# Autodesk Inventor assembly: 2024-000
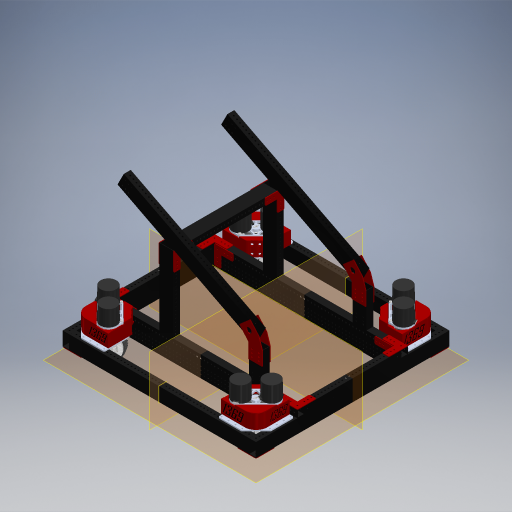
[picture p0: Inventor's stored thumbnail of the model, 512x512]
Saved by Autodesk Inventor 2024.2 (Build 282272000, 272)
## iProperties
Created: 2024-01-07
Part Number: 2024-000
Document SubType Name: Assembly
Designer: rohan
Author: rohan
## Documents named in this file (4)
- C:\Users\rohan\OneDrive - Hillsborough County Public Schools\Robotics\FIRST-Robotics-Competition\Crescendo\Minotaur-Crescendo-Robot\2024-000.iam
- C:\Users\rohan\OneDrive - Hillsborough County Public Schools\Robotics\FIRST-Robotics-Competition\Crescendo\Minotaur-Crescendo-Robot\Swerve-Drivetrain.iam
- C:\Users\rohan\OneDrive - Hillsborough County Public Schools\Robotics\FIRST-Robotics-Competition\Crescendo\Minotaur-Crescendo-Robot\Structure\Superstructure\Angle-Shootaur\2024-210-Angle-Shootaur.iam
- C:\Users\rohan\OneDrive - Hillsborough County Public Schools\Robotics\FIRST-Robotics-Competition\Crescendo\Minotaur-Crescendo-Robot\Structure\Superstructure\Angle-Shootaur\2024-220-Hard-Stop.iam
## Components (3 placed, 3 different names)
1. Swerve-Drivetrain:1 [sub-assembly] — Mate:1, Mate:2, Flush:1, Flush:2, Flush:3, Flush:4
2. 2024-210-Angle-Shootaur:1 [sub-assembly] — Mate:2, Flush:1, Flush:4
3. 2024-220-Hard-Stop:1 [sub-assembly] — Mate:1, Flush:2, Flush:3
## Relationships (6: Flush 4, Mate 2)
- Mate:1: Swerve-Drivetrain:1 ↔ 2024-220-Hard-Stop:1
- Mate:2: Swerve-Drivetrain:1 ↔ 2024-210-Angle-Shootaur:1
- Flush:1: Swerve-Drivetrain:1 ↔ 2024-210-Angle-Shootaur:1
- Flush:2: Swerve-Drivetrain:1 ↔ 2024-220-Hard-Stop:1
- Flush:3 (203.2 mm): Swerve-Drivetrain:1 ↔ 2024-220-Hard-Stop:1
- Flush:4 (127 mm): Swerve-Drivetrain:1 ↔ 2024-210-Angle-Shootaur:1
